# Autodesk Inventor assembly: MacroKeypad
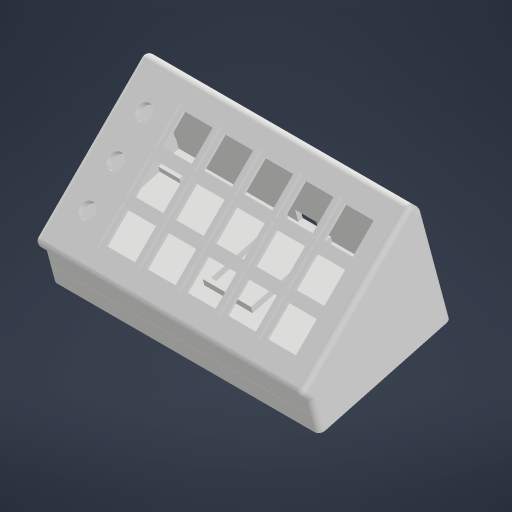
[picture p0: Inventor's stored thumbnail of the model, 512x512]
Saved by Autodesk Inventor 2024.3 (Build 283343000, 343)
## iProperties
Created: 2026-02-02
Part Number: MacroKeypad
Document SubType Name: Assembly
Designer: zokur
Author: zokur
## Documents named in this file (3)
- C:\Users\zokur\Desktop\Macro Keypad\model\MacroKeypad.iam
- C:\Users\zokur\Desktop\Macro Keypad\model\KeypadBase.ipt
- C:\Users\zokur\Desktop\Macro Keypad\model\keypadTop.ipt
## Components (2 placed, 2 different names)
1. KeypadBase:1 — Mate:1, Flush:1, Mate:2
2. keypadTop:1 — Mate:1, Flush:1, Mate:2
## Relationships (3: Mate 2, Flush 1)
- Mate:1: KeypadBase:1 ↔ keypadTop:1
- Flush:1: KeypadBase:1 ↔ keypadTop:1
- Mate:2: KeypadBase:1 ↔ keypadTop:1
